# Autodesk Inventor assembly: TorsoPelvisUnit
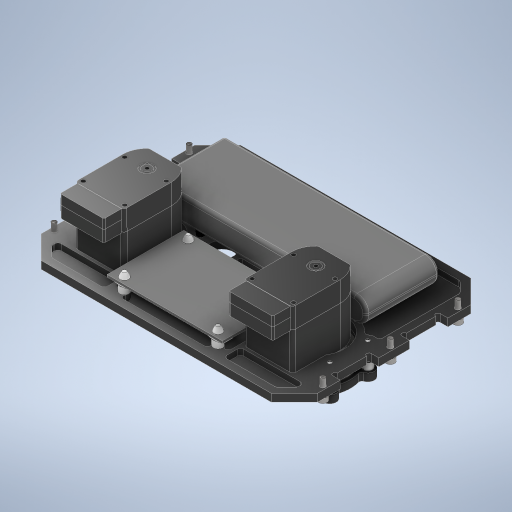
[picture p0: Inventor's stored thumbnail of the model, 512x512]
Saved by Autodesk Inventor 2024.2 (Build 282272000, 272)
## iProperties
Created: 2024-01-05
Part Number: TorsoPelvisUnit
Document SubType Name: Assembly
Designer: Masato Kubotera
Mass: 796.863 g
Surface Area: 1429.36 cm^2
Volume: 306.795 cm^3
Author: Masato Kubotera
## Documents named in this file (9)
- D:\OneDrive - Chiba Institute of Technology\CIT Brains\RoboCup2024\Mechanic\SUSTAINA-OP2-DEV - 作業\NativeFiles\Boby\Torso\TorsoPelvis\TorsoPelvisUnit.iam
- D:\OneDrive - Chiba Institute of Technology\CIT Brains\RoboCup2024\Mechanic\SUSTAINA-OP2-DEV - 作業\NativeFiles\Boby\Torso\TorsoPelvis\TorsoPelvisLowerFrame.ipt
- D:\OneDrive - Chiba Institute of Technology\CIT Brains\RoboCup2024\Mechanic\SUSTAINA-OP2-DEV - 作業\NativeFiles\Boby\CommonDesignedComponents\CrossRollerBearingUnit\CrossRollerBearingUnit.iam
- D:\OneDrive - Chiba Institute of Technology\CIT Brains\RoboCup2024\Mechanic\SUSTAINA-OP2-DEV - 作業\NativeFiles\Boby\COTS\Screws\CapScrew\UC-0310.ipt
- D:\OneDrive - Chiba Institute of Technology\CIT Brains\RoboCup2024\Mechanic\SUSTAINA-OP2-DEV - 作業\NativeFiles\Boby\COTS\Screws\CapScrew\FC-2615EB.ipt
- D:\OneDrive - Chiba Institute of Technology\CIT Brains\RoboCup2024\Mechanic\SUSTAINA-OP2-DEV - 作業\NativeFiles\Boby\COTS\Spacers\WBN-305.ipt
- D:\OneDrive - Chiba Institute of Technology\CIT Brains\RoboCup2024\Mechanic\SUSTAINA-OP2-DEV - 作業\NativeFiles\Boby\CustomElectronicComponents\SUSTAINA-POWER-INPUT-BORAD.ipt
- D:\OneDrive - Chiba Institute of Technology\CIT Brains\RoboCup2024\Mechanic\SUSTAINA-OP2-DEV - 作業\NativeFiles\Boby\COTS\Actuators\PMX-SCR-9203HV.ipt
- D:\OneDrive - Chiba Institute of Technology\CIT Brains\RoboCup2024\Mechanic\SUSTAINA-OP2-DEV - 作業\NativeFiles\Boby\COTS\ElectronicComponents\Batteries\Lipo-3250-3S-Pack-3.ipt
## Components (22 placed, 8 different names)
1. CrossRollerBearingUnit:1 [sub-assembly] — Insert:1, Insert:2
2. CrossRollerBearingUnit:2 [sub-assembly] — Insert:42, Insert:43
3. Lipo-3250-3S-Pack-3:2 — Mate:1, Mate:2, Flush:4
4. TorsoPelvisLowerFrame:1 — Flush:1, Flush:2, Flush:3, Insert:1, Insert:2, Insert:3, Insert:4, Insert:5, Insert:6, Insert:7, Insert:8, Insert:9, Insert:38, Insert:39, Insert:40, Insert:41, Insert:42, Insert:43, Insert:44, Insert:45, Insert:46, Insert:73, Insert:74, Insert:75, Insert:76, Flush:4
5. SUSTAINA-POWER-INPUT-BORAD:1 — Insert:81, Insert:82, Insert:83, Insert:84
6. PMX-SCR-9203HV:2 — Insert:3, Insert:4
7. PMX-SCR-9203HV:1 — Insert:38, Insert:39
8. Lipo-3250-3S-Pack-3:1
9. UC-0310:1 — Insert:5
10. UC-0310:2 — Insert:6
11. UC-0310:3 — Insert:7
12. UC-0310:4 — Insert:44
13. UC-0310:5 — Insert:45
14. UC-0310:6 — Insert:46
15. FC-2615EB:1 — Insert:8
16. FC-2615EB:2 — Insert:9
17. FC-2615EB:3 — Insert:40
18. FC-2615EB:4 — Insert:41
19. WBN-305:1 — Angle:1, Insert:73, Insert:81
20. WBN-305:2 — Angle:2, Insert:74, Insert:82
21. WBN-305:3 — Angle:3, Insert:75, Insert:83
22. WBN-305:4 — Angle:4, Insert:76, Insert:84
## Relationships (36: Insert 26, Flush 4, Angle 4, Mate 2)
- Flush:1: TorsoPelvisLowerFrame:1
- Flush:2: TorsoPelvisLowerFrame:1
- Flush:3: TorsoPelvisLowerFrame:1
- Insert:1: CrossRollerBearingUnit:1 ↔ TorsoPelvisLowerFrame:1
- Insert:2: CrossRollerBearingUnit:1 ↔ TorsoPelvisLowerFrame:1
- Insert:3: TorsoPelvisLowerFrame:1 ↔ PMX-SCR-9203HV:2
- Insert:4: TorsoPelvisLowerFrame:1 ↔ PMX-SCR-9203HV:2
- Insert:5: TorsoPelvisLowerFrame:1 ↔ UC-0310:1
- Insert:6: TorsoPelvisLowerFrame:1 ↔ UC-0310:2
- Insert:7: TorsoPelvisLowerFrame:1 ↔ UC-0310:3
- Insert:8: TorsoPelvisLowerFrame:1 ↔ FC-2615EB:1
- Insert:9: TorsoPelvisLowerFrame:1 ↔ FC-2615EB:2
- Insert:38: TorsoPelvisLowerFrame:1 ↔ PMX-SCR-9203HV:1
- Insert:39: TorsoPelvisLowerFrame:1 ↔ PMX-SCR-9203HV:1
- Insert:40: TorsoPelvisLowerFrame:1 ↔ FC-2615EB:3
- Insert:41: TorsoPelvisLowerFrame:1 ↔ FC-2615EB:4
- Insert:42: CrossRollerBearingUnit:2 ↔ TorsoPelvisLowerFrame:1
- Insert:43: CrossRollerBearingUnit:2 ↔ TorsoPelvisLowerFrame:1
- Insert:44: TorsoPelvisLowerFrame:1 ↔ UC-0310:4
- Insert:45: TorsoPelvisLowerFrame:1 ↔ UC-0310:5
- Insert:46: TorsoPelvisLowerFrame:1 ↔ UC-0310:6
- Angle:1 (0 deg): WBN-305:1
- Angle:2 (0 deg): WBN-305:2
- Angle:3 (0 deg): WBN-305:3
- Angle:4 (0 deg): WBN-305:4
- Insert:73: TorsoPelvisLowerFrame:1 ↔ WBN-305:1
- Insert:74: TorsoPelvisLowerFrame:1 ↔ WBN-305:2
- Insert:75: TorsoPelvisLowerFrame:1 ↔ WBN-305:3
- Insert:76: TorsoPelvisLowerFrame:1 ↔ WBN-305:4
- Insert:81: SUSTAINA-POWER-INPUT-BORAD:1 ↔ WBN-305:1
- Insert:82: SUSTAINA-POWER-INPUT-BORAD:1 ↔ WBN-305:2
- Insert:83: SUSTAINA-POWER-INPUT-BORAD:1 ↔ WBN-305:3
- Insert:84: SUSTAINA-POWER-INPUT-BORAD:1 ↔ WBN-305:4
- Mate:1: Lipo-3250-3S-Pack-3:2
- Mate:2: Lipo-3250-3S-Pack-3:2
- Flush:4: Lipo-3250-3S-Pack-3:2 ↔ TorsoPelvisLowerFrame:1
